# Autodesk Inventor assembly: Full Motor Arm (1 inch) with Kornylak Wheel
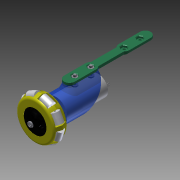
[picture p0: Inventor's stored thumbnail of the model, 180x180]
Saved by Autodesk Inventor 2014 (Build 180170000, 170)
## iProperties
Created: 2014-02-14
Part Number: Full Motor Arm (1 inch) with Kornylak Wheel
Document SubType Name: Assembly
Designer: Spooner
Author: Spooner
## Documents named in this file (8)
- C:\Users\Spooner\Documents\Inventor\FerretBall Robot\3Pod\Inventor 2014 Files\Full Motor Arm (1 inch) with Kornylak Wheel.iam
- C:\Users\Spooner\Documents\Inventor\FerretBall Robot\3Pod\Inventor 2014 Files\Flexiwheel with Hub.iam
- C:\Users\Spooner\Documents\Inventor\FerretBall Robot\3Pod\Inventor 2014 Files\Motor Mount Arm (1 inch).ipt
- C:\Users\Spooner\Documents\Inventor\FerretBall Robot\3Pod\Inventor 2014 Files\Motor Mount.ipt
- C:\Users\Spooner\Documents\Inventor\FerretBall Robot\3Pod\Inventor 2014 Files\Motor.iam
- C:\Users\Spooner\Documents\Inventor\Content Center Files\R2014\en-US\JIS B 1111(1)\JIS B 1111 - M3x10(1).ipt
- C:\Users\Spooner\Documents\Inventor\Content Center Files\R2014\en-US\JIS B 1181 U\JIS B 1181 - B M3.ipt
- C:\Users\Spooner\Documents\Inventor\Content Center Files\R2014\en-US\JIS B 1111(1)\JIS B 1111 - M3x5(1).ipt
## Components (10 placed, 7 different names)
1. Flexiwheel with Hub:1 [sub-assembly] — Insert:9
2. Motor Mount Arm (1 inch):1 — Insert:3, Mate:1, Insert:4, Insert:5, Angle:1, Angle:2
3. Motor Mount:1 — Insert:1, Insert:2, Insert:3, Insert:6, Insert:7, Insert:8
4. Motor:1 [sub-assembly] — Insert:8, Insert:9
5. JIS B 1111 M3x10:1 — Insert:2, Mate:1
6. JIS B 1111 M3x10:2 — Insert:1
7. JIS B 1181 (unchamfered) - Metric B M3:1 — Insert:4, Angle:1
8. JIS B 1181 (unchamfered) - Metric B M3:2 — Insert:5, Angle:2
9. JIS B 1111 M3x5:1 — Insert:6
10. JIS B 1111 M3x5:2 — Insert:7
## Relationships (12: Insert 9, Angle 2, Mate 1)
- Insert:1: Motor Mount:1 ↔ JIS B 1111 M3x10:2
- Insert:2: Motor Mount:1 ↔ JIS B 1111 M3x10:1
- Insert:3: Motor Mount Arm (1 inch):1 ↔ Motor Mount:1
- Mate:1: Motor Mount Arm (1 inch):1 ↔ JIS B 1111 M3x10:1
- Insert:4: Motor Mount Arm (1 inch):1 ↔ JIS B 1181 (unchamfered) - Metric B M3:1
- Insert:5: Motor Mount Arm (1 inch):1 ↔ JIS B 1181 (unchamfered) - Metric B M3:2
- Angle:1 (0 deg): Motor Mount Arm (1 inch):1 ↔ JIS B 1181 (unchamfered) - Metric B M3:1
- Angle:2 (0 deg): Motor Mount Arm (1 inch):1 ↔ JIS B 1181 (unchamfered) - Metric B M3:2
- Insert:6: Motor Mount:1 ↔ JIS B 1111 M3x5:1
- Insert:7: Motor Mount:1 ↔ JIS B 1111 M3x5:2
- Insert:8: Motor Mount:1 ↔ Motor:1
- Insert:9: Flexiwheel with Hub:1 ↔ Motor:1
